# Autodesk Inventor assembly: Wire tension assembly
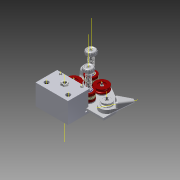
[picture p0: Inventor's stored thumbnail of the model, 180x180]
Saved by Autodesk Inventor 2013 (Build 170138000, 138)
## iProperties
Created: 2012-11-12
Part Number: Wire tension assembly
Document SubType Name: Assembly
Designer: Nico
Mass: 313.424 g
Surface Area: 1025.66 cm^2
Volume: 254.041 cm^3
Density: 1.23375 g/cm^3
Author: Nico
## Documents named in this file (23)
- D:\Documents\Inventor\Coil winder\IAM files\Wire tension assembly.iam
- D:\Documents\Inventor\Coil winder\IPT files\Wire guidance base assembly.ipt
- D:\Documents\Inventor\Coil winder\IPT files\Washer M3 nickel plated.ipt
- D:\Documents\Inventor\Coil winder\IPT files\felt.ipt
- D:\Documents\Inventor\Coil winder\IPT files\Nut M4 nickel plated.ipt
- D:\Documents\Inventor\Coil winder\IPT files\Nut M3 nickel plated.ipt
- D:\Documents\Inventor\Coil winder\Wire tension assembly\Design Accelerator\Compress Spring1.iam
- D:\Documents\Inventor\Coil winder\IPT files\M4 Carre Washer Nickel plated.ipt
- D:\Documents\Inventor\Coil winder\IPT files\M4 Washer Nickel plated.ipt
- D:\Documents\Inventor\Coil winder\IPT files\Tension knob.ipt
- D:\Documents\Inventor\Coil winder\IPT files\Tension Push washer.ipt
- D:\Documents\Inventor\Coil winder\IPT files\Nut M3 Torque nickel plated.ipt
- D:\Documents\Inventor\Coil winder\IPT files\bolt M3 x 30 nickel plated.ipt
- D:\Documents\Inventor\Coil winder\IPT files\bolt M3 x 25 nickel plated.ipt
- D:\Documents\Inventor\Coil winder\IPT files\Tension Push washer backplate.ipt
- D:\Documents\Inventor\Coil winder\IAM files\wire guidance wheel.iam
- D:\Documents\Inventor\Coil winder\IAM files\wire guidance.iam
- D:\Documents\Inventor\Coil winder\IPT files\lineair bearing 8 x15 x 24.ipt
- D:\Documents\Inventor\Coil winder\IPT files\Nut M8.ipt
- D:\Documents\Inventor\Coil winder\IPT files\bolt M3 x 20 nickel plated.ipt
- D:\Documents\Inventor\Coil winder\IPT files\bolt M3 x 16 nickel plated.ipt
- D:\Documents\Inventor\Coil winder\IPT files\carriage.ipt
- D:\Documents\Inventor\Coil winder\IPT files\bolt M4 x 70 nickel plated.ipt
## Components (62 placed, 23 different names)
1. wire guidance wheel:2 [sub-assembly] — Mate:120, Mate:121, Mate:122
2. Wire guidance base assembly:1 — Mate:93, Mate:94, Mate:96, Mate:103, Mate:104, Mate:105, Mate:106, Mate:115, Mate:116, Mate:118, Mate:120, Mate:124, Mate:126, Mate:127, Mate:130, Mate:133, Mate:138, Mate:139, Mate:156, Mate:159, Mate:222, Mate:225, Mate:228, Mate:239, Mate:240, Mate:241, Mate:242
3. felt:1 — Mate:20, Mate:98, Mate:248
4. bolt M3 x 25 nickel plated:1 — Mate:89, Mate:90, Mate:94, Mate:117
5. Washer M3 Nickel plated:2 — Mate:104
6. felt:2 — Mate:20, Mate:51, Mate:100
7. Compress Spring:1 [sub-assembly] — Mate:25, Flush:3, Mate:102
8. M4 Carre Washer nickel plated:1 — Mate:23, Flush:3, Mate:30, Mate:31, Mate:32
9. M4 Carre Washer nickel plated:2 — Mate:23, Mate:25, Mate:52, Mate:101
10. Bolt M4 x 70 nickel plated:1 — Mate:27, Mate:28, Mate:50, Mate:96, Mate:98, Mate:100, Mate:101, Mate:102, Mate:123, Mate:246
11. M4 Washer nickel plated:1 — Mate:27, Mate:28, Mate:103
12. Tension knob:1 — Mate:30, Mate:31, Mate:33
13. Nut M4 nickel plated:2 — Mate:32, Mate:33
14. Tension Push washer:1 — Mate:50, Mate:51, Mate:52
15. Nut M3 nickel plated:2 — Mate:132, Mate:134, Mate:135
16. Nut M3 Torque nickel plated:1 — Mate:122
17. bolt M3 x 30 nickel plated:1 — Mate:127, Mate:128, Mate:129, Mate:131, Mate:132, Mate:136
18. Washer M3 Nickel plated:6 — Mate:131, Mate:133, Mate:134
19. Nut M3 Torque nickel plated:2 — Mate:111, Mate:112
20. Nut M3 nickel plated:4 — Mate:107, Mate:108, Mate:110
21. Nut M3 nickel plated:6 — Mate:90, Mate:119, Mate:121
22. Washer M3 Nickel plated:7 — Mate:89
23. wire guidance wheel:1 [sub-assembly] — Mate:93, Mate:109, Mate:110, Mate:111, Mate:112
24. Washer M3 Nickel plated:8 — Mate:105, Mate:106, Mate:107, Mate:108, Mate:109
25. bolt M3 x 25 nickel plated:2 — Mate:113, Mate:114, Mate:115
26. Washer M3 Nickel plated:9 — Mate:113, Mate:114, Mate:116
27. Washer M3 Nickel plated:10 — Mate:117, Mate:118, Mate:119
28. Washer M3 Nickel plated:11 — Mate:128, Mate:129, Mate:130
29. Tension Push washer backplate:1 — Mate:123, Mate:124, Mate:247, Mate:248
30. wire guidance:1 [sub-assembly] — Mate:126, Mate:135, Mate:137
31. Nut M3 nickel plated:7 — Mate:136, Mate:137
32. Tension Push washer backplate:2 — Mate:138, Mate:139, Mate:140, Mate:141, Mate:244, Mate:245
33. felt:3 — Mate:140, Mate:143, Mate:245
34. felt:4 — Mate:141, Mate:143, Mate:144, Mate:145
35. Tension Push washer:2 — Mate:144, Mate:145, Mate:146, Mate:147, Mate:148
36. M4 Carre Washer nickel plated:3 — Mate:150, Mate:151, Mate:154
37. M4 Carre Washer nickel plated:4 — Mate:146, Mate:147, Mate:149
38. Tension knob:2 — Mate:152, Mate:154, Mate:155
39. Compress Spring:2 [sub-assembly] — Mate:148, Mate:149, Mate:150, Mate:151, Mate:152, Mate:153
40. Nut M4 nickel plated:3 — Mate:153, Mate:155
41. Bolt M4 x 10 nickel plated:4 — Mate:156, Mate:157, Mate:158, Mate:243
42. M4 Washer nickel plated:2 — Mate:157, Mate:158, Mate:159
43. lineair bearing 8 x15 x 24:1 — Mate:223, Mate:234
44. lineair bearing 8 x15 x 24:2 — Mate:224, Mate:233
45. Nut M8:1 — Mate:227, Mate:232
46. Bolt M3 x 20 nickel plated:1 — Mate:180, Mate:182
47. Bolt M3 x 20 nickel plated:2 — Mate:181, Mate:183
48. Bolt M3 x 16 nickel plated:1 — Mate:172, Mate:174
49. Bolt M3 x 16 nickel plated:2 — Mate:173, Mate:175
50. Washer M3 Nickel plated:12 — Mate:172, Mate:174
51. Washer M3 Nickel plated:13 — Mate:173, Mate:175
52. Washer M3 Nickel plated:14 — Mate:180, Mate:182
53. Washer M3 Nickel plated:15 — Mate:181, Mate:183, Mate:226
54. Compress Spring:3 [sub-assembly] — Mate:221, Mate:229, Mate:230, Mate:231
55. Nut M8:2 — Mate:221, Mate:231
56. carriage:1 — Mate:222, Mate:223, Mate:224, Mate:225, Mate:226, Mate:227, Mate:228, Mate:229, Mate:230, Mate:232, Mate:233, Mate:234, Mate:235, Mate:236, Mate:237, Mate:238
57. Nut M3 nickel plated:8 — Mate:235, Mate:240
58. Nut M3 nickel plated:9 — Mate:236, Mate:242
59. Nut M3 nickel plated:10 — Mate:238, Mate:241
60. Nut M3 nickel plated:11 — Mate:237, Mate:239
61. Nut M4 nickel plated:4 — Mate:243, Mate:244
62. Nut M4 nickel plated:5 — Mate:246, Mate:247
## Relationships (117: Mate 116, Flush 1)
- [Mate]: bolt M3 x 25 nickel plated:1 ↔ Washer M3 Nickel plated:2
- [Mate]: bolt M3 x 25 nickel plated:1 ↔ Washer M3 Nickel plated:2
- Mate:20 (0.5 mm): felt:1 ↔ felt:2
- Mate:23: M4 Carre Washer nickel plated:1 ↔ M4 Carre Washer nickel plated:2
- Mate:25: Compress Spring:1 ↔ M4 Carre Washer nickel plated:2
- Flush:3: Compress Spring:1 ↔ M4 Carre Washer nickel plated:1
- Mate:27: Bolt M4 x 70 nickel plated:1 ↔ M4 Washer nickel plated:1
- Mate:28: Bolt M4 x 70 nickel plated:1 ↔ M4 Washer nickel plated:1
- Mate:30: M4 Carre Washer nickel plated:1 ↔ Tension knob:1
- Mate:31: M4 Carre Washer nickel plated:1 ↔ Tension knob:1
- Mate:32: M4 Carre Washer nickel plated:1 ↔ Nut M4 nickel plated:2
- Mate:33: Tension knob:1 ↔ Nut M4 nickel plated:2
- Mate:50: Bolt M4 x 70 nickel plated:1 ↔ Tension Push washer:1
- Mate:51: felt:2 ↔ Tension Push washer:1
- Mate:52: M4 Carre Washer nickel plated:2 ↔ Tension Push washer:1
- [Mate]: bolt M3 x 25 nickel plated:1 ↔ Nut M3 Torque nickel plated:1
- [Mate]: bolt M3 x 25 nickel plated:1 ↔ Washer M3 Nickel plated:7
- Mate:89: bolt M3 x 25 nickel plated:1 ↔ Washer M3 Nickel plated:7
- Mate:90: bolt M3 x 25 nickel plated:1 ↔ Nut M3 nickel plated:6
- Mate:93: Wire guidance base assembly:1 ↔ wire guidance wheel:1
- Mate:94: Wire guidance base assembly:1 ↔ bolt M3 x 25 nickel plated:1
- Mate:96: Wire guidance base assembly:1 ↔ Bolt M4 x 70 nickel plated:1
- Mate:98: felt:1 ↔ Bolt M4 x 70 nickel plated:1
- Mate:100: felt:2 ↔ Bolt M4 x 70 nickel plated:1
- Mate:101: M4 Carre Washer nickel plated:2 ↔ Bolt M4 x 70 nickel plated:1
- Mate:102: Compress Spring:1 ↔ Bolt M4 x 70 nickel plated:1
- Mate:103: Wire guidance base assembly:1 ↔ M4 Washer nickel plated:1
- Mate:104: Wire guidance base assembly:1 ↔ Washer M3 Nickel plated:2
- Mate:105: Wire guidance base assembly:1 ↔ Washer M3 Nickel plated:8
- Mate:106: Wire guidance base assembly:1 ↔ Washer M3 Nickel plated:8
- Mate:107: Nut M3 nickel plated:4 ↔ Washer M3 Nickel plated:8
- Mate:108: Nut M3 nickel plated:4 ↔ Washer M3 Nickel plated:8
- Mate:109: wire guidance wheel:1 ↔ Washer M3 Nickel plated:8
- Mate:110: Nut M3 nickel plated:4 ↔ wire guidance wheel:1
- Mate:111: Nut M3 Torque nickel plated:2 ↔ wire guidance wheel:1
- Mate:112: Nut M3 Torque nickel plated:2 ↔ wire guidance wheel:1
- Mate:113: bolt M3 x 25 nickel plated:2 ↔ Washer M3 Nickel plated:9
- Mate:114: bolt M3 x 25 nickel plated:2 ↔ Washer M3 Nickel plated:9
- Mate:115: Wire guidance base assembly:1 ↔ bolt M3 x 25 nickel plated:2
- Mate:116: Wire guidance base assembly:1 ↔ Washer M3 Nickel plated:9
- Mate:117: bolt M3 x 25 nickel plated:1 ↔ Washer M3 Nickel plated:10
- Mate:118: Wire guidance base assembly:1 ↔ Washer M3 Nickel plated:10
- Mate:119: Nut M3 nickel plated:6 ↔ Washer M3 Nickel plated:10
- Mate:120: wire guidance wheel:2 ↔ Wire guidance base assembly:1
- Mate:121: wire guidance wheel:2 ↔ Nut M3 nickel plated:6
- Mate:122: wire guidance wheel:2 ↔ Nut M3 Torque nickel plated:1
- Mate:123: Bolt M4 x 70 nickel plated:1 ↔ Tension Push washer backplate:1
- Mate:124: Wire guidance base assembly:1 ↔ Tension Push washer backplate:1
- Mate:126: Wire guidance base assembly:1 ↔ wire guidance:1
- Mate:127: Wire guidance base assembly:1 ↔ bolt M3 x 30 nickel plated:1
- Mate:128: bolt M3 x 30 nickel plated:1 ↔ Washer M3 Nickel plated:11
- Mate:129: bolt M3 x 30 nickel plated:1 ↔ Washer M3 Nickel plated:11
- Mate:130: Wire guidance base assembly:1 ↔ Washer M3 Nickel plated:11
- Mate:131: bolt M3 x 30 nickel plated:1 ↔ Washer M3 Nickel plated:6
- Mate:132: Nut M3 nickel plated:2 ↔ bolt M3 x 30 nickel plated:1
- Mate:133: Wire guidance base assembly:1 ↔ Washer M3 Nickel plated:6
- Mate:134: Nut M3 nickel plated:2 ↔ Washer M3 Nickel plated:6
- Mate:135: Nut M3 nickel plated:2 ↔ wire guidance:1
- Mate:136: bolt M3 x 30 nickel plated:1 ↔ Nut M3 nickel plated:7
- Mate:137: wire guidance:1 ↔ Nut M3 nickel plated:7
- Mate:138: Wire guidance base assembly:1 ↔ Tension Push washer backplate:2
- Mate:139: Wire guidance base assembly:1 ↔ Tension Push washer backplate:2
- Mate:140: Tension Push washer backplate:2 ↔ felt:3
- Mate:141: Tension Push washer backplate:2 ↔ felt:4
- Mate:143 (0.5 mm): felt:3 ↔ felt:4
- Mate:144: felt:4 ↔ Tension Push washer:2
- Mate:145: felt:4 ↔ Tension Push washer:2
- Mate:146: Tension Push washer:2 ↔ M4 Carre Washer nickel plated:4
- Mate:147: Tension Push washer:2 ↔ M4 Carre Washer nickel plated:4
- Mate:148: Tension Push washer:2 ↔ Compress Spring:2
- Mate:149: M4 Carre Washer nickel plated:4 ↔ Compress Spring:2
- Mate:150: M4 Carre Washer nickel plated:3 ↔ Compress Spring:2
- Mate:151: M4 Carre Washer nickel plated:3 ↔ Compress Spring:2
- Mate:152: Tension knob:2 ↔ Compress Spring:2
- Mate:153: Compress Spring:2 ↔ Nut M4 nickel plated:3
- Mate:154: M4 Carre Washer nickel plated:3 ↔ Tension knob:2
- Mate:155: Tension knob:2 ↔ Nut M4 nickel plated:3
- Mate:156: Wire guidance base assembly:1 ↔ Bolt M4 x 10 nickel plated:4
- Mate:157: Bolt M4 x 10 nickel plated:4 ↔ M4 Washer nickel plated:2
- Mate:158: Bolt M4 x 10 nickel plated:4 ↔ M4 Washer nickel plated:2
- Mate:159: Wire guidance base assembly:1 ↔ M4 Washer nickel plated:2
- Mate:172: Bolt M3 x 16 nickel plated:1 ↔ Washer M3 Nickel plated:12
- Mate:173: Bolt M3 x 16 nickel plated:2 ↔ Washer M3 Nickel plated:13
- Mate:174: Bolt M3 x 16 nickel plated:1 ↔ Washer M3 Nickel plated:12
- Mate:175: Bolt M3 x 16 nickel plated:2 ↔ Washer M3 Nickel plated:13
- Mate:180: Bolt M3 x 20 nickel plated:1 ↔ Washer M3 Nickel plated:14
- Mate:181: Bolt M3 x 20 nickel plated:2 ↔ Washer M3 Nickel plated:15
- Mate:182: Bolt M3 x 20 nickel plated:1 ↔ Washer M3 Nickel plated:14
- Mate:183: Bolt M3 x 20 nickel plated:2 ↔ Washer M3 Nickel plated:15
- Mate:221: Compress Spring:3 ↔ Nut M8:2
- Mate:222: Wire guidance base assembly:1 ↔ carriage:1
- Mate:223: lineair bearing 8 x15 x 24:1 ↔ carriage:1
- Mate:224: lineair bearing 8 x15 x 24:2 ↔ carriage:1
- Mate:225: Wire guidance base assembly:1 ↔ carriage:1
- Mate:226: Washer M3 Nickel plated:15 ↔ carriage:1
- Mate:227: Nut M8:1 ↔ carriage:1
- Mate:228: Wire guidance base assembly:1 ↔ carriage:1
- Mate:229: Compress Spring:3 ↔ carriage:1
- Mate:230: Compress Spring:3 ↔ carriage:1
- Mate:231: Compress Spring:3 ↔ Nut M8:2
- Mate:232: Nut M8:1 ↔ carriage:1
- Mate:233: lineair bearing 8 x15 x 24:2 ↔ carriage:1
- Mate:234: lineair bearing 8 x15 x 24:1 ↔ carriage:1
- Mate:235: carriage:1 ↔ Nut M3 nickel plated:8
- Mate:236: carriage:1 ↔ Nut M3 nickel plated:9
- Mate:237: carriage:1 ↔ Nut M3 nickel plated:11
- Mate:238: carriage:1 ↔ Nut M3 nickel plated:10
- Mate:239: Wire guidance base assembly:1 ↔ Nut M3 nickel plated:11
- Mate:240: Wire guidance base assembly:1 ↔ Nut M3 nickel plated:8
- Mate:241: Wire guidance base assembly:1 ↔ Nut M3 nickel plated:10
- Mate:242: Wire guidance base assembly:1 ↔ Nut M3 nickel plated:9
- Mate:243: Bolt M4 x 10 nickel plated:4 ↔ Nut M4 nickel plated:4
- Mate:244: Tension Push washer backplate:2 ↔ Nut M4 nickel plated:4
- Mate:245: Tension Push washer backplate:2 ↔ felt:3
- Mate:246: Bolt M4 x 70 nickel plated:1 ↔ Nut M4 nickel plated:5
- Mate:247: Tension Push washer backplate:1 ↔ Nut M4 nickel plated:5
- Mate:248: felt:1 ↔ Tension Push washer backplate:1
